# Autodesk Inventor assembly: Gripper
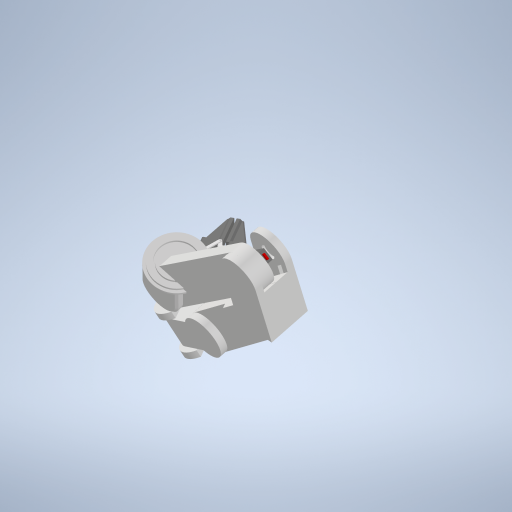
[picture p0: Inventor's stored thumbnail of the model, 512x512]
Saved by Autodesk Inventor 2023 (Build 270158000, 158)
## iProperties
Created: 2024-06-26
Part Number: Gripper
Document SubType Name: Assembly
Designer: Swoby
Author: Swoby
## Documents named in this file (17)
- C:\Users\Swoby\OneDrive\Plocha\DUM-E\V0.3\Gripper.iam
- C:\Users\Swoby\OneDrive\Plocha\DUM-E\V0.3\gripper_head.ipt
- C:\Users\Swoby\OneDrive\Plocha\DUM-E\V0.3\gripper_gripper.ipt
- C:\Users\Swoby\OneDrive\Plocha\DUM-E\V0.3\gripper_mechanism2.ipt
- C:\Users\Swoby\OneDrive\Plocha\DUM-E\V0.3\Servo_small_maketa.ipt
- C:\Users\Swoby\OneDrive\Plocha\DUM-E\V0.3\wirst 1 right.ipt
- C:\Users\Swoby\OneDrive\Plocha\DUM-E\V0.3\wirst 2 right.ipt
- C:\Users\Swoby\OneDrive\Plocha\DUM-E\V0.3\Servo_bigg_maketa.ipt
- C:\Users\Swoby\OneDrive\Plocha\DUM-E\V0.3\Servo_bigg_top.ipt
- C:\Users\Swoby\OneDrive\Plocha\DUM-E\V0.3\arm 1 right.ipt
- C:\Users\Swoby\OneDrive\Plocha\DUM-E\V0.3\wirst 2 left.ipt
- C:\Users\Swoby\OneDrive\Plocha\DUM-E\V0.3\arm 1 leftt.ipt
- C:\Users\Swoby\OneDrive\Plocha\DUM-E\V0.3\arm 2 right.ipt
- C:\Users\Swoby\OneDrive\Plocha\DUM-E\V0.3\Base 1 left.ipt
- C:\Users\Swoby\OneDrive\Plocha\DUM-E\V0.3\Base 1 right.ipt
- C:\Users\Swoby\OneDrive\Plocha\DUM-E\V0.3\Servo_small_top.ipt
- C:\Users\Swoby\OneDrive\Plocha\DUM-E\V0.3\gripper_mechanism.ipt
## Components (26 placed, 16 different names)
1. gripper_head:1 — Mate:1, Mate:2, Mate:3, Mate:4, Mate:20, Mate:21, Mate:22, Mate:26, Mate:27
2. gripper_gripper:1 — Mate:1, Mate:4, Mate:10, Mate:64
3. gripper_gripper:2 — Mate:2, Mate:3, Mate:9, Mate:65
4. gripper_mechanism2:1 — Mate:10, Mate:64, Mate:69
5. gripper_mechanism2:2 — Mate:9, Mate:65, Mate:68
6. Servo_small_maketa:2 — Mate:20, Mate:21, Mate:22, Mate:62, Mate:63
7. wirst 1 right:1 — Mate:28, Mate:29, Mate:30, Mate:36, Mate:37
8. wirst 2 right:1 — Mate:33, Mate:34, Mate:35, Mate:43, Mate:44, Mate:45, Flush:1, Flush:2
9. Servo_bigg_maketa:1 — Mate:31, Mate:32, Mate:33, Mate:34, Mate:35
10. Servo_bigg_maketa:2 — Mate:24, Mate:25, Mate:28, Mate:29, Mate:30
11. Servo_bigg_top:1 — Mate:31, Mate:32, Mate:36, Mate:37
12. Servo_bigg_top:2 — Mate:24, Mate:25, Mate:26, Mate:27
13. arm 1 right:1 — Mate:38, Mate:39, Mate:40, Mate:46, Flush:3, Flush:4, Mate:57, Mate:58
14. Servo_bigg_maketa:3 — Mate:38, Mate:39, Mate:40, Mate:41, Mate:42
15. Servo_bigg_top:3 — Mate:41, Mate:42, Mate:43, Mate:44
16. wirst 2 left:1 — Mate:45, Flush:1, Flush:2
17. arm 1 leftt:1 — Mate:46, Flush:3, Flush:4
18. arm 2 right:1 — Mate:51, Mate:52, Mate:53, Mate:54, Mate:55, Mate:56
19. Servo_bigg_top:4 — Mate:47, Mate:49, Mate:57, Mate:58
20. Servo_bigg_top:5 — Mate:48, Mate:50, Mate:60, Mate:61
21. Servo_bigg_maketa:4 — Mate:48, Mate:50, Mate:51, Mate:52, Mate:53
22. Servo_bigg_maketa:5 — Mate:47, Mate:49, Mate:54, Mate:55, Mate:56
23. Base 1 left:1 — Mate:59, Flush:5, Flush:6, Mate:60, Mate:61
24. Base 1 right:1 — Mate:59, Flush:5, Flush:6
25. Servo_small_top:1 — Mate:62, Mate:63, Mate:66, Mate:67, Mate:70
26. gripper_mechanism:1 — Mate:66, Mate:67, Mate:68, Mate:69, Mate:70
## Relationships (62: Mate 56, Flush 6)
- Mate:1: gripper_head:1 ↔ gripper_gripper:1
- Mate:2: gripper_head:1 ↔ gripper_gripper:2
- Mate:3: gripper_head:1 ↔ gripper_gripper:2
- Mate:4: gripper_head:1 ↔ gripper_gripper:1
- Mate:9: gripper_gripper:2 ↔ gripper_mechanism2:2
- Mate:10: gripper_gripper:1 ↔ gripper_mechanism2:1
- Mate:20: gripper_head:1 ↔ Servo_small_maketa:2
- Mate:21: gripper_head:1 ↔ Servo_small_maketa:2
- Mate:22: gripper_head:1 ↔ Servo_small_maketa:2
- Mate:24: Servo_bigg_maketa:2 ↔ Servo_bigg_top:2
- Mate:25: Servo_bigg_maketa:2 ↔ Servo_bigg_top:2
- Mate:26: gripper_head:1 ↔ Servo_bigg_top:2
- Mate:27: gripper_head:1 ↔ Servo_bigg_top:2
- Mate:28: wirst 1 right:1 ↔ Servo_bigg_maketa:2
- Mate:29: wirst 1 right:1 ↔ Servo_bigg_maketa:2
- Mate:30: wirst 1 right:1 ↔ Servo_bigg_maketa:2
- Mate:31: Servo_bigg_maketa:1 ↔ Servo_bigg_top:1
- Mate:32: Servo_bigg_maketa:1 ↔ Servo_bigg_top:1
- Mate:33: wirst 2 right:1 ↔ Servo_bigg_maketa:1
- Mate:34: wirst 2 right:1 ↔ Servo_bigg_maketa:1
- Mate:35: wirst 2 right:1 ↔ Servo_bigg_maketa:1
- Mate:36: wirst 1 right:1 ↔ Servo_bigg_top:1
- Mate:37: wirst 1 right:1 ↔ Servo_bigg_top:1
- Mate:38: arm 1 right:1 ↔ Servo_bigg_maketa:3
- Mate:39: arm 1 right:1 ↔ Servo_bigg_maketa:3
- Mate:40: arm 1 right:1 ↔ Servo_bigg_maketa:3
- Mate:41: Servo_bigg_maketa:3 ↔ Servo_bigg_top:3
- Mate:42: Servo_bigg_maketa:3 ↔ Servo_bigg_top:3
- Mate:43: wirst 2 right:1 ↔ Servo_bigg_top:3
- Mate:44: wirst 2 right:1 ↔ Servo_bigg_top:3
- Mate:45: wirst 2 right:1 ↔ wirst 2 left:1
- Flush:1: wirst 2 right:1 ↔ wirst 2 left:1
- Flush:2: wirst 2 right:1 ↔ wirst 2 left:1
- Mate:46: arm 1 right:1 ↔ arm 1 leftt:1
- Flush:3: arm 1 right:1 ↔ arm 1 leftt:1
- Flush:4: arm 1 right:1 ↔ arm 1 leftt:1
- Mate:47: Servo_bigg_top:4 ↔ Servo_bigg_maketa:5
- Mate:48: Servo_bigg_top:5 ↔ Servo_bigg_maketa:4
- Mate:49: Servo_bigg_top:4 ↔ Servo_bigg_maketa:5
- Mate:50: Servo_bigg_top:5 ↔ Servo_bigg_maketa:4
- Mate:51: arm 2 right:1 ↔ Servo_bigg_maketa:4
- Mate:52: arm 2 right:1 ↔ Servo_bigg_maketa:4
- Mate:53: arm 2 right:1 ↔ Servo_bigg_maketa:4
- Mate:54: arm 2 right:1 ↔ Servo_bigg_maketa:5
- Mate:55: arm 2 right:1 ↔ Servo_bigg_maketa:5
- Mate:56: arm 2 right:1 ↔ Servo_bigg_maketa:5
- Mate:57: arm 1 right:1 ↔ Servo_bigg_top:4
- Mate:58: arm 1 right:1 ↔ Servo_bigg_top:4
- Mate:59: Base 1 left:1 ↔ Base 1 right:1
- Flush:5: Base 1 left:1 ↔ Base 1 right:1
- Flush:6: Base 1 left:1 ↔ Base 1 right:1
- Mate:60: Servo_bigg_top:5 ↔ Base 1 left:1
- Mate:61: Servo_bigg_top:5 ↔ Base 1 left:1
- Mate:62: Servo_small_maketa:2 ↔ Servo_small_top:1
- Mate:63: Servo_small_maketa:2 ↔ Servo_small_top:1
- Mate:64: gripper_gripper:1 ↔ gripper_mechanism2:1
- Mate:65: gripper_gripper:2 ↔ gripper_mechanism2:2
- Mate:66: Servo_small_top:1 ↔ gripper_mechanism:1
- Mate:67: Servo_small_top:1 ↔ gripper_mechanism:1
- Mate:68: gripper_mechanism2:2 ↔ gripper_mechanism:1
- Mate:69: gripper_mechanism2:1 ↔ gripper_mechanism:1
- Mate:70: Servo_small_top:1 ↔ gripper_mechanism:1
